# Autodesk Inventor assembly: Torso
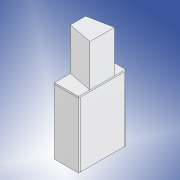
[picture p0: Inventor's stored thumbnail of the model, 180x180]
Saved by Autodesk Inventor 2017 (Build 210142000, 142)
## iProperties
Created: 2017-06-21
Part Number: Torso
Document SubType Name: Assembly
Designer: zallen
Author: zallen
## Documents named in this file (5)
- C:\Users\zallen\Documents\GitHub\cr-laundry-robot\src\Body 2\Torso Assembly\Torso.iam
- C:\Users\zallen\Documents\GitHub\cr-laundry-robot\src\Body 2\Torso Assembly\TA001.ipt
- C:\Users\zallen\Documents\GitHub\cr-laundry-robot\src\Body 2\Torso Assembly\TA002.ipt
- C:\Users\zallen\Documents\GitHub\cr-laundry-robot\src\Body 2\Torso Assembly\TA003.ipt
- C:\Users\zallen\Documents\GitHub\cr-laundry-robot\src\Body 2\Torso Assembly\TA004.ipt
## Components (6 placed, 4 different names)
1. TA001:1 — Mate:1, Mate:2, Mate:5, Mate:6
2. TA002:1 — Mate:1, Mate:2, Mate:3, Mate:4, Mate:9
3. TA001:2 — Mate:3, Mate:4, Mate:7, Mate:8
4. TA002:2 — Mate:5, Mate:6, Mate:7
5. TA003:1 — Mate:8, Mate:9, Mate:10, Mate:11
6. TA004:1 — Mate:10, Mate:11
## Relationships (11: Mate 11)
- Mate:1: TA001:1 ↔ TA002:1
- Mate:2: TA001:1 ↔ TA002:1
- Mate:3: TA002:1 ↔ TA001:2
- Mate:4: TA002:1 ↔ TA001:2
- Mate:5: TA001:1 ↔ TA002:2
- Mate:6: TA001:1 ↔ TA002:2
- Mate:7: TA001:2 ↔ TA002:2
- Mate:8: TA001:2 ↔ TA003:1
- Mate:9: TA002:1 ↔ TA003:1
- Mate:10: TA003:1 ↔ TA004:1
- Mate:11: TA003:1 ↔ TA004:1
